# Autodesk Inventor assembly: Arm
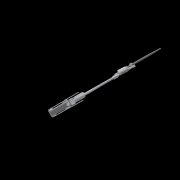
[picture p0: Inventor's stored thumbnail of the model, 180x180]
Saved by Autodesk Inventor 2020 (Build 240168000, 168)
## iProperties
Created: 2020-03-24
Part Number: Arm
Document SubType Name: Assembly
Designer: valer
Mass: 4853.13 g
Surface Area: 3141.52 cm^2
Volume: 1403.99 cm^3
Density: 3.45667 g/cm^3
Author: valer
## Documents named in this file (16)
- C:\Users\valer\Desktop\drumming-robot\src\Arm.iam
- C:\Users\valer\Desktop\drumming-robot\src\UpperArm.ipt
- C:\Users\valer\Desktop\drumming-robot\src\UpperArmBracket.ipt
- C:\Users\valer\Desktop\drumming-robot\src\Forearm.ipt
- C:\Users\valer\Desktop\drumming-robot\src\external\Drumstick.ipt
- C:\Users\valer\Desktop\drumming-robot\src\external\ForearmShaftCollar.ipt
- C:\Users\valer\Desktop\drumming-robot\src\external\PushSolenoid.ipt
- C:\Users\valer\Desktop\drumming-robot\src\external\UpperArmActuatorBody.ipt
- C:\Users\valer\Desktop\drumming-robot\src\external\UpperArmActuatorShaft.ipt
- C:\Users\valer\Desktop\drumming-robot\src\external\ForearmActuatorBody.ipt
- C:\Users\valer\Desktop\drumming-robot\src\external\ForearmActuatorShaft.ipt
- C:\Users\valer\Desktop\drumming-robot\src\ForearmActuatorConnector.ipt
- C:\Users\valer\Desktop\drumming-robot\src\UpperArmBracketMirror.ipt
- C:\Users\valer\Desktop\drumming-robot\src\UpperArmActuatorBracket.ipt
- C:\Users\valer\Desktop\drumming-robot\src\UpperArmActuatorBracketMirror.ipt
- C:\Users\valer\Desktop\drumming-robot\src\UpperArmMount.ipt
## Components (16 placed, 15 different names)
1. Drumstick:1 — Mate:79, Flush:3
2. ShaftCollar1/2:1 — Mate:79, Flush:3, Mate:236, Flush:18, Mate:275
3. PushSolenoid:1 — Mate:274, Mate:275
4. UpperArmActuatorBody:1 — Mate:257, Mate:266
5. Forearm:1 — Flush:17, Mate:227, Mate:236, Flush:18, Mate:239, Mate:244, Mate:274
6. UpperArmActuatorShaft:2 — Mate:238, Flush:20, Mate:266
7. ForearmActuatorBody:1 — Mate:231, Mate:232, Mate:234, Flush:19
8. ForearmActuatorShaft:3 — Flush:17, Mate:231, Mate:232, Mate:241, Mate:243, Angle:10, Mate:246
9. UpperArm:3 — Mate:227, Mate:234, Mate:238, Flush:19, Flush:20, Mate:248, Mate:249, Mate:263, Mate:264, Mate:265
10. ForearmActuatorConnector:1 — Mate:239, Mate:241, Mate:245, Angle:10, Mate:246
11. ForearmActuatorConnector:2 — Mate:243, Mate:244, Mate:245
12. UpperArmBracket:5 — Mate:249, Mate:254, Mate:255, Mate:256, Flush:21, Mate:265, Mate:267, Mate:272
13. UpperArmBracketMirror:1 — Mate:248, Mate:251, Mate:252, Mate:253, Flush:21, Mate:263, Mate:264, Mate:270, Mate:271
14. UpperArmActuatorBracket:1 — Mate:254, Mate:255, Mate:256, Mate:262
15. UpperArmActuatorBracketMirror:1 — Mate:251, Mate:252, Mate:253, Mate:257
16. UpperArmMount:1 — Mate:267, Mate:270, Mate:271, Mate:272, Mate:273
## Relationships (41: Mate 34, Flush 6, Angle 1)
- Mate:79: Drumstick:1 ↔ ShaftCollar1/2:1
- Flush:3 (304.8 mm): Drumstick:1 ↔ ShaftCollar1/2:1
- Flush:17: Forearm:1 ↔ ForearmActuatorShaft:3
- Mate:227: Forearm:1 ↔ UpperArm:3
- Mate:231: ForearmActuatorBody:1 ↔ ForearmActuatorShaft:3
- Mate:232: ForearmActuatorBody:1 ↔ ForearmActuatorShaft:3
- Mate:234: ForearmActuatorBody:1 ↔ UpperArm:3
- Mate:236: ShaftCollar1/2:1 ↔ Forearm:1
- Flush:18 (12.7 mm): ShaftCollar1/2:1 ↔ Forearm:1
- Mate:238: UpperArmActuatorShaft:2 ↔ UpperArm:3
- Flush:19: ForearmActuatorBody:1 ↔ UpperArm:3
- Flush:20: UpperArmActuatorShaft:2 ↔ UpperArm:3
- Mate:239: Forearm:1 ↔ ForearmActuatorConnector:1
- Mate:241: ForearmActuatorShaft:3 ↔ ForearmActuatorConnector:1
- Mate:243: ForearmActuatorShaft:3 ↔ ForearmActuatorConnector:2
- Mate:244: Forearm:1 ↔ ForearmActuatorConnector:2
- Mate:245: ForearmActuatorConnector:1 ↔ ForearmActuatorConnector:2
- Angle:10 (-180 deg): ForearmActuatorShaft:3 ↔ ForearmActuatorConnector:1
- Mate:246: ForearmActuatorShaft:3 ↔ ForearmActuatorConnector:1
- Mate:248: UpperArm:3 ↔ UpperArmBracketMirror:1
- Mate:249: UpperArm:3 ↔ UpperArmBracket:5
- Mate:251: UpperArmBracketMirror:1 ↔ UpperArmActuatorBracketMirror:1
- Mate:252: UpperArmBracketMirror:1 ↔ UpperArmActuatorBracketMirror:1
- Mate:253: UpperArmBracketMirror:1 ↔ UpperArmActuatorBracketMirror:1
- Mate:254: UpperArmBracket:5 ↔ UpperArmActuatorBracket:1
- Mate:255: UpperArmBracket:5 ↔ UpperArmActuatorBracket:1
- Mate:256: UpperArmBracket:5 ↔ UpperArmActuatorBracket:1
- Flush:21: UpperArmBracket:5 ↔ UpperArmBracketMirror:1
- Mate:257: UpperArmActuatorBody:1 ↔ UpperArmActuatorBracketMirror:1
- Mate:262: UpperArmActuatorBracket:1
- Mate:263: UpperArm:3 ↔ UpperArmBracketMirror:1
- Mate:264: UpperArm:3 ↔ UpperArmBracketMirror:1
- Mate:265: UpperArm:3 ↔ UpperArmBracket:5
- Mate:266: UpperArmActuatorBody:1 ↔ UpperArmActuatorShaft:2
- Mate:267: UpperArmBracket:5 ↔ UpperArmMount:1
- Mate:270: UpperArmBracketMirror:1 ↔ UpperArmMount:1
- Mate:271: UpperArmBracketMirror:1 ↔ UpperArmMount:1
- Mate:272: UpperArmBracket:5 ↔ UpperArmMount:1
- Mate:273: UpperArmMount:1
- Mate:274: PushSolenoid:1 ↔ Forearm:1
- Mate:275 (25.4 mm): ShaftCollar1/2:1 ↔ PushSolenoid:1
